# Autodesk Inventor assembly: turret_assembly
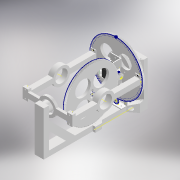
[picture p0: Inventor's stored thumbnail of the model, 180x180]
Saved by Autodesk Inventor 2021 (Build 250183000, 183)
## iProperties
Created: 2020-09-03
Part Number: turret_assembly
Document SubType Name: Assembly
Designer: bober
Author: bober
## Documents named in this file (12)
- C:\Turret\Turret\Models\turret_assembly.iam
- C:\Turret\Turret\Models\turret_assembly\Design Accelerator\vertical_axis_small_gear.ipt
- C:\Turret\Turret\Models\turret_assembly\Design Accelerator\vertical_axis_bigl_gear.ipt
- C:\Turret\Turret\Models\turret_assembly\Design Accelerator\horizontal_axis_big_gear.ipt
- C:\Turret\Turret\Models\turret_assembly\Design Accelerator\pylon.ipt
- C:\Turret\Turret\Models\turret_assembly\Design Accelerator\upper_grip.ipt
- C:\Turret\Turret\Models\turret_assembly\Design Accelerator\main_stand_lower_half.ipt
- C:\Turret\Turret\Models\turret_assembly\Design Accelerator\main_stand_upper_half.ipt
- C:\Turret\Turret\Models\step_motor\Nema 17 Motor a Pasos 17HS4401.iam
- C:\Turret\Turret\Models\turret_assembly\Design Accelerator\horizontal_lower_bearing_holder.ipt
- C:\Turret\Turret\Models\turret_assembly\Design Accelerator\horizontal_axis_motor_metal_holder.ipt
- C:\Turret\Turret\Models\turret_assembly\Design Accelerator\vertical_axis_motor_metal_holder.ipt
## Components (14 placed, 11 different names)
1. vertical_axis_small_gear:1 — Rigid:4
2. horizontal_axis_big_gear:1 — Rotational:5
3. vertical_axis_small_gear:2
4. vertical_axis_bigl_gear:2 — Rigid:2, Rigid:3, Rotational:6, Rotational:7
5. pylon:1 — Rigid:2
6. pylon:2 — Rigid:3, Rotational:1, Rotational:5
7. upper_grip:1 — Rotational:1
8. main_stand_lower_half:1 — Rotational:4, Rigid:5, Flush:1
9. main_stand_upper_half:1 — Rotational:4
10. Nema 17 Motor a Pasos 17HS4401:2 [sub-assembly] — Rigid:4
11. Nema 17 Motor a Pasos 17HS4401:3 [sub-assembly] — Rotational:8
12. horizontal_lower_bearing_holder:1 — Rotational:6, Flush:1
13. horizontal_axis_motor_metal_holder:1 — Rotational:7, Rotational:8
14. vertical_axis_motor_metal_holder:1 — Rigid:5
## Relationships (11: RevoluteJoint 6, WeldJoint 4, Flush 1)
- Rigid:2 [WeldJoint]: vertical_axis_bigl_gear:2 ↔ pylon:1
- Rigid:3 [WeldJoint]: vertical_axis_bigl_gear:2 ↔ pylon:2
- Rotational:1 [RevoluteJoint]: pylon:2 ↔ upper_grip:1
- Rotational:4 [RevoluteJoint]: main_stand_lower_half:1 ↔ main_stand_upper_half:1
- Rotational:5 [RevoluteJoint] (-52.75 mm): horizontal_axis_big_gear:1 ↔ pylon:2
- Rigid:4 [WeldJoint]: vertical_axis_small_gear:1 ↔ Nema 17 Motor a Pasos 17HS4401:2
- Rotational:6 [RevoluteJoint]: vertical_axis_bigl_gear:2 ↔ horizontal_lower_bearing_holder:1
- Rotational:7 [RevoluteJoint]: vertical_axis_bigl_gear:2 ↔ horizontal_axis_motor_metal_holder:1
- Rotational:8 [RevoluteJoint]: Nema 17 Motor a Pasos 17HS4401:3 ↔ horizontal_axis_motor_metal_holder:1
- Rigid:5 [WeldJoint]: main_stand_lower_half:1 ↔ vertical_axis_motor_metal_holder:1
- Flush:1: main_stand_lower_half:1 ↔ horizontal_lower_bearing_holder:1
